# Autodesk Inventor assembly: Assembly1
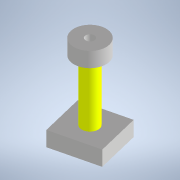
[picture p0: Inventor's stored thumbnail of the model, 180x180]
Saved by Autodesk Inventor 2021 (Build 250183000, 183)
## iProperties
Created: 2023-05-09
Part Number: Assembly1
Document SubType Name: Assembly
Designer: assman
Author: assman
## Documents named in this file (3)
- C:\dev\3DModels\3party\daisq\Assembly1.iam
- C:\dev\3DModels\3party\daisq\pieza1.ipt
- C:\dev\3DModels\3party\daisq\pieza2.ipt
## Components (2 placed, 2 different names)
1. pieza1:1 — Rotational:1
2. pieza2:1 — Rotational:1
## Relationships (1: RevoluteJoint 1)
- Rotational:1 [RevoluteJoint] (-0.5 mm): pieza1:1 ↔ pieza2:1
